# Autodesk Inventor assembly: Assembly_Cube_empty_IM_v3
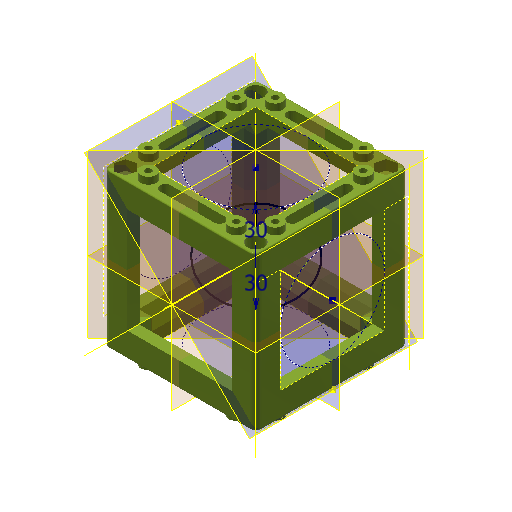
[picture p0: Inventor's stored thumbnail of the model, 512x512]
Saved by Autodesk Inventor 2022 (Build 260153000, 153)
## iProperties
Created: 2020-03-27
Part Number: Assembly_Cube_empty_IM_v3
Document SubType Name: Assembly
Designer: B
Author: B
## Documents named in this file (2)
- C:\Users\diederichbenedict\Dropbox\Dokumente\Promotion\PROJECTS\UC2\02_CAD\INVENTOR\uc2_v3\Assembly_Cube_empty_IM_v3.iam
- C:\Users\diederichbenedict\Dropbox\Dokumente\Promotion\PROJECTS\UC2\02_CAD\INVENTOR\uc2_v3\10_Cube_1x1_IM.ipt
## Components (2 placed, 1 different names)
1. 10_Cube_1x1_IM:1 — Mate:1, Angle:1, Mate:2, Symmetry:1, Passend:3, Winkel:2, Symmetrie:2, Symmetrie:3, Symmetrie:4
2. 10_Cube_1x1_IM:2 — Flush:1, Flush:2, Flush:3, Mate:1, Angle:1, Mate:2, Symmetry:1, Symmetrie:2, Symmetrie:3, Symmetrie:4
## Relationships (12: Symmetry 4, Flush 3, Mate 3, Angle 2)
- Flush:1: 10_Cube_1x1_IM:2
- Flush:2: 10_Cube_1x1_IM:2
- Flush:3: 10_Cube_1x1_IM:2
- Mate:1: 10_Cube_1x1_IM:1 ↔ 10_Cube_1x1_IM:2
- Angle:1 (0 deg): 10_Cube_1x1_IM:1 ↔ 10_Cube_1x1_IM:2
- Mate:2 (-50.1 mm): 10_Cube_1x1_IM:1 ↔ 10_Cube_1x1_IM:2
- Symmetry:1: 10_Cube_1x1_IM:1 ↔ 10_Cube_1x1_IM:2
- Passend:3 [Mate]: 10_Cube_1x1_IM:1
- Winkel:2 [Angle] (90 deg): 10_Cube_1x1_IM:1
- Symmetrie:2: 10_Cube_1x1_IM:1 ↔ 10_Cube_1x1_IM:2
- Symmetrie:3: 10_Cube_1x1_IM:1 ↔ 10_Cube_1x1_IM:2
- Symmetrie:4: 10_Cube_1x1_IM:1 ↔ 10_Cube_1x1_IM:2
